# Autodesk Inventor assembly: Kolben
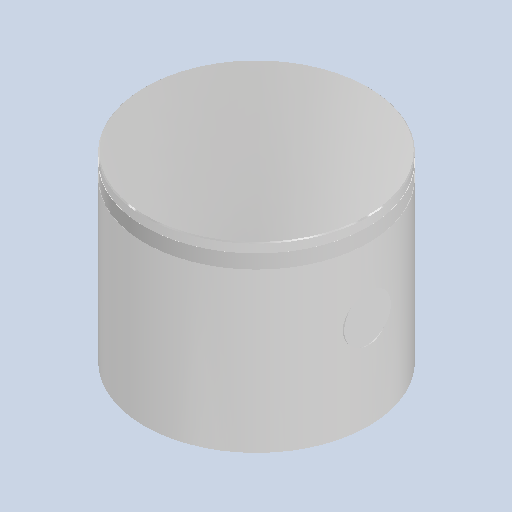
[picture p0: Inventor's stored thumbnail of the model, 512x512]
Saved by Autodesk Inventor 2025 (Build 290162010, 162A)
## iProperties
Created: 2024-07-17
Part Number: Kolben
Document SubType Name: Assembly
Designer: ffogue
Author: ffogue
## Documents named in this file (4)
- C:\Users\ffogue\OneDrive - MuM - OM\Dokumente\Inventor\Boxermotor\Kolben.iam
- C:\Users\ffogue\OneDrive - MuM - OM\Dokumente\Inventor\Boxermotor\Kolben.ipt
- C:\Users\ffogue\OneDrive - MuM - OM\Dokumente\Inventor\Boxermotor\kolbenring.ipt
- C:\Users\ffogue\OneDrive - MuM - OM\Dokumente\Inventor\Boxermotor\KolbenFitting.ipt
## Components (3 placed, 3 different names)
1. Kolben:1 — Insert:1, Cylindrical:1
2. kolbenring:1 — Insert:1
3. KolbenFitting:1 — Cylindrical:1
## Relationships (2: Insert 1, CylindricalJoint 1)
- Insert:1: Kolben:1 ↔ kolbenring:1
- Cylindrical:1: Kolben:1 ↔ KolbenFitting:1
